# Autodesk Inventor assembly: Сборка1
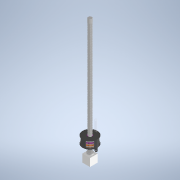
[picture p0: Inventor's stored thumbnail of the model, 180x180]
Saved by Autodesk Inventor 2021 (Build 250183000, 183)
## iProperties
Created: 2022-06-28
Part Number: Сборка1
Document SubType Name: Assembly
Designer: termi
Mass: 4018.46 g
Surface Area: 5918.73 cm^2
Volume: 3467.81 cm^3
Density: 1.15879 g/cm^3
Author: termi
## Documents named in this file (11)
- C:\Users\termi\OneDrive\Документы\Inventor\Projects\Mecanical amplifier\Сборка1.iam
- C:\Users\termi\OneDrive\Документы\Inventor\Projects\Mecanical amplifier\main screw.ipt
- C:\Users\termi\OneDrive\Документы\Inventor\Projects\Mecanical amplifier\right nut.ipt
- C:\Users\termi\OneDrive\Документы\Inventor\Projects\Mecanical amplifier\left nut.ipt
- C:\Users\termi\OneDrive\Документы\Inventor\Projects\Mecanical amplifier\motor.ipt
- C:\Users\termi\OneDrive\Документы\Inventor\Projects\Mecanical amplifier\1.ipt
- C:\Users\termi\OneDrive\Документы\Inventor\Projects\Mecanical amplifier\inner_part.ipt
- C:\Users\termi\OneDrive\Документы\Inventor\Projects\Mecanical amplifier\Сборка1\Мастер проектирования\Подшипник4.iam
- C:\Users\termi\OneDrive\Документы\Inventor\Projects\Mecanical amplifier\2.ipt
- C:\Users\termi\OneDrive\Документы\Inventor\Content Center Files\R2021\ru-RU\ISO 4762(2)\ISO 4762 - M4 x 40ISO.ipt
- C:\Users\termi\OneDrive\Документы\Inventor\Projects\Mecanical amplifier\outer_part.ipt
## Components (15 placed, 10 different names)
1. main screw:1 — С поворотом:1, Совмещение:1, Совмещение:2, Совмещение:3, Угол:1, Совмещение:4, Угол:2, Угол:3, Угол:6
2. right nut:1 — Совмещение:2, Совмещение:3, Угол:1, Жесткий:2
3. left nut:1 — Совмещение:1, Совмещение:4, Угол:2, Жесткий:1
4. motor:1 — С поворотом:1, Угол:6
5. 1:1 — Жесткий:1, С поворотом:2
6. 2:1 — Жесткий:2, Совмещение:5, Заподлицо:11
7. inner_part:1 — Заподлицо:10, С поворотом:3, Угол:4, С поворотом:4, Угол:5, Совмещение:6, Совмещение:7, Цилиндрический:1, Заподлицо:12
8. Подшипник:1 [sub-assembly] — Совмещение:5, Заподлицо:11, Угол:3
9. Подшипник:2 [sub-assembly] — С поворотом:2, С поворотом:3, Угол:4
10. Подшипник:3 [sub-assembly] — С поворотом:4, Угол:5
11. outer_part:1 — Цилиндрический:1, Заподлицо:12
12. ISO 4762 M4 x 40:1 — Совмещение:6, Совмещение:7
13. ISO 4762 M4 x 40:2
14. ISO 4762 M4 x 40:3
15. ISO 4762 M4 x 40:4
## Component patterns: (4 elements, first: ISO 4762 M4 x 40:1)
## Relationships (23: Mate 7, Angle 6, RevoluteJoint 4, Flush 3, WeldJoint 2, CylindricalJoint 1)
- С поворотом:1 [RevoluteJoint]: main screw:1 ↔ motor:1
- Совмещение:1 [Mate]: main screw:1 ↔ left nut:1
- Совмещение:2 [Mate]: main screw:1 ↔ right nut:1
- Угол:1 [Angle] (1178.4 deg): main screw:1 ↔ right nut:1
- Совмещение:4 [Mate] (141.2 mm): main screw:1 ↔ left nut:1
- Угол:2 [Angle]: main screw:1 ↔ left nut:1
- Жесткий:1 [WeldJoint]: left nut:1 ↔ 1:1
- Жесткий:2 [WeldJoint]: right nut:1 ↔ 2:1
- Совмещение:3 [Mate] (98.2 mm): main screw:1 ↔ right nut:1
- Заподлицо:10 [Flush]: inner_part:1
- Совмещение:5 [Mate]: 2:1 ↔ Подшипник:1
- Заподлицо:11 [Flush]: 2:1 ↔ Подшипник:1
- Угол:3 [Angle] (-258 deg): main screw:1 ↔ Подшипник:1
- С поворотом:2 [RevoluteJoint]: 1:1 ↔ Подшипник:2
- С поворотом:3 [RevoluteJoint]: inner_part:1 ↔ Подшипник:2
- Угол:4 [Angle]: inner_part:1 ↔ Подшипник:2
- С поворотом:4 [RevoluteJoint]: inner_part:1 ↔ Подшипник:3
- Угол:5 [Angle] (-802.2 deg): inner_part:1 ↔ Подшипник:3
- Угол:6 [Angle] (49 deg): main screw:1 ↔ motor:1
- Совмещение:6 [Mate]: inner_part:1 ↔ ISO 4762 M4 x 40:1
- Совмещение:7 [Mate]: inner_part:1 ↔ ISO 4762 M4 x 40:1
- Цилиндрический:1 [CylindricalJoint]: inner_part:1 ↔ outer_part:1
- Заподлицо:12 [Flush]: inner_part:1 ↔ outer_part:1
